# Autodesk Inventor assembly: Assembly5_Pantalla_LCD_20x4_Completo
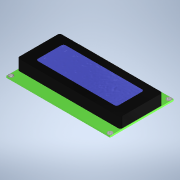
[picture p0: Inventor's stored thumbnail of the model, 180x180]
Saved by Autodesk Inventor 2021 (Build 250183000, 183)
## iProperties
Created: 2022-06-26
Part Number: Assembly5_Pantalla_LCD_20x4_Completo
Document SubType Name: Assembly
Designer: Sam14
Author: Sam14
## Documents named in this file (4)
- C:\Users\Tecneu\Documents\ZD\Modelos 3D\Pantalla LCD + I2C\Assembly5_Pantalla_LCD_20x4_Completo.iam
- C:\Users\Tecneu\Documents\ZD\Modelos 3D\Pantalla LCD + I2C\Part1_Pantalla_LCD_20x4.ipt
- C:\Users\Tecneu\Documents\ZD\Modelos 3D\Pantalla LCD + I2C\Interfaz_I2C.iam
- C:\Users\Tecneu\Documents\ZD\Modelos 3D\Pantalla LCD + I2C\Jumper2.ipt
## Components (3 placed, 3 different names)
1. Part1_Pantalla_LCD_20x4:1 — Flush:1, Flush:2, Flush:3, Mate:1, Mate:2, Flush:4
2. Interfaz_I2C:1 [sub-assembly] — Mate:1, Mate:2, Flush:4, Mate:3, Flush:5, Mate:4, Flush:6
3. Jumper2:1 — Mate:3, Flush:5, Mate:4, Flush:6
## Relationships (10: Flush 6, Mate 4)
- Flush:1: Part1_Pantalla_LCD_20x4:1
- Flush:2: Part1_Pantalla_LCD_20x4:1
- Flush:3: Part1_Pantalla_LCD_20x4:1
- Mate:1: Part1_Pantalla_LCD_20x4:1 ↔ Interfaz_I2C:1
- Mate:2: Part1_Pantalla_LCD_20x4:1 ↔ Interfaz_I2C:1
- Flush:4 (-2.54 mm): Part1_Pantalla_LCD_20x4:1 ↔ Interfaz_I2C:1
- Mate:3: Interfaz_I2C:1 ↔ Jumper2:1
- Flush:5 (1 mm): Interfaz_I2C:1 ↔ Jumper2:1
- Mate:4: Interfaz_I2C:1 ↔ Jumper2:1
- Flush:6 (2.5 mm): Interfaz_I2C:1 ↔ Jumper2:1
